# Autodesk Inventor assembly: писюны_MIR
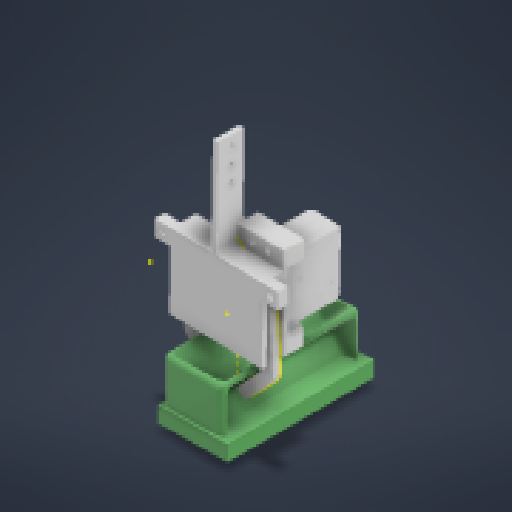
[picture p0: Inventor's stored thumbnail of the model, 512x512]
Saved by Autodesk Inventor 2025 (Build 290162000, 162)
## iProperties
Created: 2024-12-28
Part Number: писюны_MIR
Document SubType Name: Assembly
Designer: GameHD
Author: Phantom
## Documents named in this file (7)
- C:\Users\GameHD\Desktop\phantom 16950\писюны_MIR.iam
- C:\Users\GameHD\Desktop\phantom 16950\am-5401 Sample_MIR.ipt
- C:\Users\GameHD\Downloads\Telegram Desktop\Клешни с фиксатором\Клешни с фиксатором_MIR.ipt
- C:\Users\GameHD\Desktop\phantom 16950\писюн 2_MIR1.ipt
- C:\Users\GameHD\Desktop\phantom 16950\писюн_MIR.ipt
- C:\Users\GameHD\Desktop\phantom 16950\держать писюны_MIR.ipt
- C:\Users\GameHD\Desktop\phantom 16950\2000-0025-0002\2000-0025-0002_MIR3.ipt
## Components (8 placed, 6 different names)
1. am-5401 Sample_MIR:1
2. Клешни с фиксатором_MIR:1
3. писюн 2_MIR1:1
4. писюн_MIR:1
5. писюн 2_MIR1:2 — Совмещение:1, Заподлицо:1, Совмещение:4, Совмещение:5
6. писюн_MIR:2 — Заподлицо:1, Совмещение:2
7. держать писюны_MIR:1 — Совмещение:4, Совмещение:6
8. 2000-0025-0002_MIR3:1 — Совмещение:6, Совмещение:5
## Relationships (6: Mate 5, Flush 1)
- Совмещение:1 [Mate]: писюн 2_MIR1:2
- Заподлицо:1 [Flush]: писюн 2_MIR1:2 ↔ писюн_MIR:2
- Совмещение:2 [Mate]: писюн_MIR:2
- Совмещение:4 [Mate]: писюн 2_MIR1:2 ↔ держать писюны_MIR:1
- Совмещение:6 [Mate]: держать писюны_MIR:1 ↔ 2000-0025-0002_MIR3:1
- Совмещение:5 [Mate]: писюн 2_MIR1:2 ↔ 2000-0025-0002_MIR3:1
